# Autodesk Inventor assembly: opener
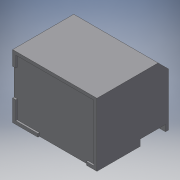
[picture p0: Inventor's stored thumbnail of the model, 180x180]
Saved by Autodesk Inventor 2018 (Build 220112000, 112)
## iProperties
Created: 2018-06-27
Part Number: opener
Document SubType Name: Assembly
Designer: erwin
Author: erwin
## Documents named in this file (3)
- D:\Erwin\OneDrive\Dualog\Hackathon2018\design\opener.iam
- D:\Erwin\OneDrive\Dualog\Hackathon2018\design\case.ipt
- D:\Erwin\OneDrive\Dualog\Hackathon2018\design\cap.ipt
## Components (2 placed, 2 different names)
1. case:1 — Flush:1, Flush:2
2. cap:1 — Flush:1, Flush:2
## Relationships (2: Flush 2)
- Flush:1: case:1 ↔ cap:1
- Flush:2: case:1 ↔ cap:1
